# Autodesk Inventor assembly: Assembly1
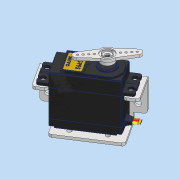
[picture p0: Inventor's stored thumbnail of the model, 180x180]
Saved by Autodesk Inventor 2021.4 (Build 254397000, 397)
## iProperties
Created: 2022-08-25
Part Number: Assembly1
Document SubType Name: Assembly
Designer: ferbm
Author: ferbm
## Documents named in this file (4)
- C:\Users\ferbm\Documents\Inventor\Projects\NuevoRobot\Assembly1.iam
- C:\Users\ferbm\Documents\Inventor\Projects\NuevoRobot\MG995.ipt
- C:\Users\ferbm\Documents\Inventor\Projects\NuevoRobot\Soporte MULTIUSOS.ipt
- C:\Users\ferbm\Documents\Inventor\Projects\NuevoRobot\MG995_Gear2.ipt
## Components (3 placed, 3 different names)
1. MG995:1 — Mate:1, Mate:2, Insert:1, Insert:2
2. Soporte MULTIUSOS:1 — Mate:1, Mate:2, Insert:1
3. MG995_Gear2:1 — Insert:2
## Relationships (4: Mate 2, Insert 2)
- Mate:1: MG995:1 ↔ Soporte MULTIUSOS:1
- Mate:2: MG995:1 ↔ Soporte MULTIUSOS:1
- Insert:1: MG995:1 ↔ Soporte MULTIUSOS:1
- Insert:2: MG995:1 ↔ MG995_Gear2:1
